# Autodesk Inventor assembly: 6P Sprocket
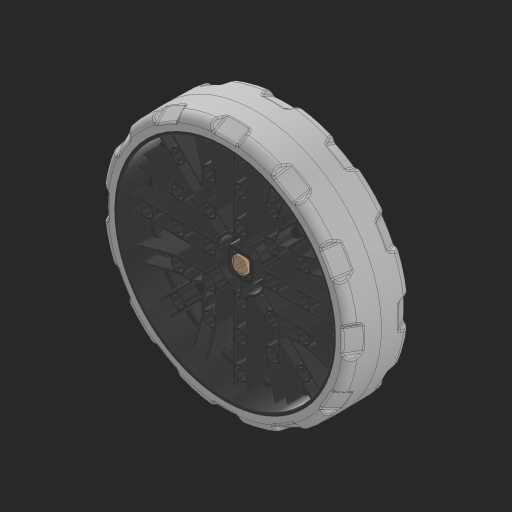
[picture p0: Inventor's stored thumbnail of the model, 512x512]
Saved by Autodesk Inventor 2023 (Build 270158000, 158)
## iProperties
Created: 2022-08-02
Part Number: 6P Sprocket
Document SubType Name: Assembly
Designer: ylu12
Author: ylu12
## Documents named in this file (3)
- C:\Users\ylu12\Documents\GitHub\VEX-CAD-Inventor\Motion\Wheels\Traction Wheel\4 Traction AS, No Insert.iam
- C:\Users\ylu12\Documents\GitHub\VEX-CAD-Inventor\Motion\Wheels\Reference Files\4 Traction Antistatic.ipt
- C:\Users\ylu12\Documents\GitHub\VEX-CAD-Inventor\Motion\Wheels\Traction Wheel.iam
## Components (1 placed, 1 different names)
1. 4 Traction Antistatic:1 — Mate:21, Mate:23, Mate:25
## Relationships (3: Mate 3)
- Mate:21: 4 Traction Antistatic:1
- Mate:23: 4 Traction Antistatic:1
- Mate:25: 4 Traction Antistatic:1
## Named parameters: Thickness = 8.255 mm
